# Autodesk Inventor assembly: Assembly_Cube_Lens_Cylindrical_v3
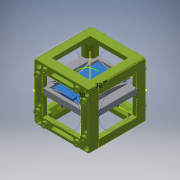
[picture p0: Inventor's stored thumbnail of the model, 180x180]
Saved by Autodesk Inventor 2019 (Build 230136000, 136)
## iProperties
Created: 2019-07-23
Part Number: Assembly_Cube_Lens_Cylindrical_v3
Document SubType Name: Assembly
Designer: marsikovabarbora
Mass: 41.9543 g
Surface Area: 260.494 cm^2
Volume: 37.9382 cm^3
Density: 1.10586 g/cm^3
Author: marsikovabarbora
## Documents named in this file (4)
- C:\Users\marsikovabarbora\Dropbox\UC2\02_CAD\INVENTOR\uc2_v3\Assembly_Cube_Lens_Cylindrical_v3.iam
- C:\Users\marsikovabarbora\Dropbox\UC2\02_CAD\INVENTOR\uc2_v3\Assembly_Cube_empty_IM_v3.iam
- C:\Users\marsikovabarbora\Dropbox\UC2\02_CAD\INVENTOR\uc2_v3\20_Cube_Insert_Lens_Cylindrical_v3.ipt
- C:\Users\marsikovabarbora\Dropbox\UC2\02_CAD\INVENTOR\uc2_v3\00_Comar_Lens_Cylindrical_50mm.ipt
## Components (3 placed, 3 different names)
1. Assembly_Cube_empty_IM_v3:1 [sub-assembly] — Mate:1, Mate:2, Mate:3, Flush:1, Mate:4, Angle:1
2. 20_Cube_Insert_Lens_Cylindrical_v3:1 — Flush:1, Mate:4, Angle:1, Flush:2
3. 00_Comar_Lens_Cylindrical_50mm:1 — Flush:2
## Relationships (7: Mate 4, Flush 2, Angle 1)
- Mate:1: Assembly_Cube_empty_IM_v3:1
- Mate:2: Assembly_Cube_empty_IM_v3:1
- Mate:3: Assembly_Cube_empty_IM_v3:1
- Flush:1: Assembly_Cube_empty_IM_v3:1 ↔ 20_Cube_Insert_Lens_Cylindrical_v3:1
- Mate:4: Assembly_Cube_empty_IM_v3:1 ↔ 20_Cube_Insert_Lens_Cylindrical_v3:1
- Angle:1 (0 deg): Assembly_Cube_empty_IM_v3:1 ↔ 20_Cube_Insert_Lens_Cylindrical_v3:1
- Flush:2: 20_Cube_Insert_Lens_Cylindrical_v3:1 ↔ 00_Comar_Lens_Cylindrical_50mm:1
